# Autodesk Inventor assembly: Synchronous Belts Transmission
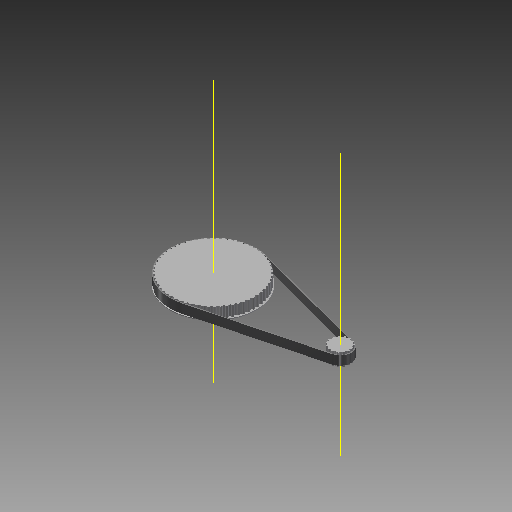
[picture p0: Inventor's stored thumbnail of the model, 512x512]
Saved by Autodesk Inventor 2018 (Build 220112000, 112)
## iProperties
ClientObjectVersion: 1
Created: 2019-11-13
Part Number: Synchronous Belts Transmission
Document SubType Name: Assembly
Designer: Bunny320
Author: Bunny320
## Documents named in this file (4)
- C:\Users\Bunny320\Desktop\sechs\4-CAD\generated\J1_belt\Design Accelerator\Synchronous Belts Transmission1.iam
- C:\Users\Bunny320\Desktop\sechs\4-CAD\generated\J1_belt\Design Accelerator\Synchronous Belt1.ipt
- C:\Users\Bunny320\Desktop\sechs\4-CAD\generated\J1_belt\Design Accelerator\Synchronous Pulley11.ipt
- C:\Users\Bunny320\Desktop\sechs\4-CAD\generated\J1_belt\Design Accelerator\Synchronous Pulley21.ipt
## Components (3 placed, 3 different names)
1. Synchronous Belt:1 — Flush:1, Mate:1, Mate:2, Flush:2, Mate:3, Mate:4
2. Synchronous Pulley1:1 — Flush:1, Mate:1, Mate:2, Rotation:1
3. Synchronous Pulley2:1 — Flush:2, Mate:3, Rotation:1, Mate:4
## Relationships (7: Mate 4, Flush 2, RelateRotation 1)
- Flush:1: Synchronous Belt:1 ↔ Synchronous Pulley1:1
- Mate:1: Synchronous Belt:1 ↔ Synchronous Pulley1:1
- Mate:2: Synchronous Belt:1 ↔ Synchronous Pulley1:1
- Flush:2: Synchronous Belt:1 ↔ Synchronous Pulley2:1
- Mate:3: Synchronous Belt:1 ↔ Synchronous Pulley2:1
- Rotation:1 [RelateRotation] (4 ul): Synchronous Pulley1:1 ↔ Synchronous Pulley2:1
- Mate:4: Synchronous Belt:1 ↔ Synchronous Pulley2:1
